# Autodesk Inventor assembly: x_motor
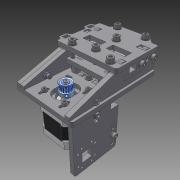
[picture p0: Inventor's stored thumbnail of the model, 180x180]
Saved by Autodesk Inventor 2014 (Build 180170000, 170)
## iProperties
Created: 2013-12-01
Part Number: x_motor
Document SubType Name: Assembly
Designer: buben
Author: buben
## Documents named in this file (23)
- C:\Users\buben\Documents\GitHub\bacon\inventor files\assemblies\x_motor.iam
- C:\Users\buben\Documents\GitHub\bacon\inventor files\printer parts\x_motor_back.ipt
- C:\Users\buben\Documents\GitHub\bacon\inventor files\printer parts\x_motor_wall_upper.ipt
- C:\Users\buben\Documents\GitHub\bacon\inventor files\printer parts\x_motor_middle.ipt
- C:\Users\buben\Documents\GitHub\bacon\inventor files\printer parts\x_motor_smooth_rod_spacer.ipt
- C:\Users\buben\Documents\GitHub\bacon\inventor files\3rd party components\linear_bearing_8\Imported Components\LU8MM\LU8MM.iam
- C:\Users\buben\Documents\GitHub\bacon\inventor files\printer parts\x_motor_top.ipt
- C:\Users\buben\Documents\GitHub\bacon\inventor files\utils\washer_m5.ipt
- C:\Users\buben\Documents\Inventor\Content Center Files\R2014\en-US\ISO 4762(2)\ISO 4762 - M5 x 45ISO.ipt
- C:\Users\buben\Documents\Inventor\Content Center Files\R2014\en-US\ISO 7040\ISO 7040 - M5.ipt
- C:\Users\buben\Documents\GitHub\bacon\inventor files\printer parts\x_motor_wall_lower.ipt
- C:\Users\buben\Documents\GitHub\bacon\inventor files\printer parts\x_motor_lower_nut_stop.ipt
- C:\Users\buben\Documents\GitHub\bacon\inventor files\utils\washer_m4.ipt
- C:\Users\buben\Documents\Inventor\Content Center Files\R2014\en-US\ISO 4762(2)\ISO 4762 - M4 x 20ISO.ipt
- C:\Users\buben\Documents\Inventor\Content Center Files\R2014\en-US\ISO 7040\ISO 7040 - M4.ipt
- C:\Users\buben\Documents\GitHub\bacon\inventor files\printer parts\x_motor_upper_nut_stop.ipt
- C:\Users\buben\Documents\Inventor\Content Center Files\R2014\en-US\ISO 4032(2)\ISO 4032 - M5ISO.ipt
- C:\Users\buben\Documents\GitHub\bacon\inventor files\printer parts\x_motor_cable_mount.ipt
- C:\Users\buben\Documents\GitHub\bacon\inventor files\printer parts\x_motor_cable_mount_brace.ipt
- C:\Users\buben\Documents\GitHub\bacon\inventor files\printer parts\motor_spacer.ipt
- C:\Users\buben\Documents\GitHub\bacon\inventor files\3rd party components\nema_17_stepper\Imported Components\NEMA 17 with T5 Pulley\NEMA 17 with T5 Pulley.iam
- C:\Users\buben\Documents\Inventor\Content Center Files\R2014\en-US\ISO 4762(2)\ISO 4762 - M3 x 20ISO.ipt
- C:\Users\buben\Documents\GitHub\bacon\inventor files\utils\washer_m3.ipt
## Components (73 placed, 22 different names)
1. x_motor_back:1 — Flush:1, Mate:1, Flush:2, Mate:2, Mate:3, Mate:4, Mate:8, Mate:9, Mate:10, Mate:11, Mate:12, Mate:13, Mate:35, Mate:36, Mate:37, Mate:38, Mate:39, Mate:40, Mate:59, Mate:60, Mate:61, Mate:77, Mate:103, Mate:104, Mate:105, Mate:109, Mate:110, Mate:113, Mate:114, Mate:130, Tangent:1, Tangent:2, Mate:131, Mate:132, Mate:133, Mate:134, Mate:139
2. x_motor_wall_upper:1 — Mate:2, Mate:3, Mate:4, Mate:5, Mate:6, Mate:7, Mate:20, Mate:21, Mate:78, Flush:3, Mate:85, Mate:100, Mate:101
3. x_motor_middle:1 — Mate:5, Mate:6, Mate:7, Mate:14, Mate:15, Mate:16, Mate:17, Mate:18, Mate:19, Mate:62, Mate:64
4. x_motor_smooth_rod_spacer:1 — Mate:8, Mate:9, Mate:10
5. x_motor_smooth_rod_spacer:2 — Mate:11, Mate:12, Mate:13
6. LU8MM:1 [sub-assembly] — Mate:14, Mate:15, Mate:18
7. LU8MM:2 [sub-assembly] — Mate:16, Mate:17, Mate:19, Mate:22
8. x_motor_top:1 — Mate:20, Mate:21, Mate:22, Mate:23, Mate:24, Mate:25, Mate:26, Mate:27, Mate:28, Mate:29, Mate:30, Mate:31, Mate:32, Mate:33, Mate:34
9. CSN 02 1702 B B 5,3:1 — Mate:26, Mate:31, Insert:1
10. CSN 02 1702 B B 5,3:2 — Mate:24, Mate:34, Insert:5
11. CSN 02 1702 B B 5,3:3 — Mate:23, Mate:32, Insert:6
12. CSN 02 1702 B B 5,3:4 — Mate:25, Mate:33, Insert:4
13. CSN 02 1702 B B 5,3:5 — Mate:27, Mate:29, Insert:3
14. CSN 02 1702 B B 5,3:6 — Mate:28, Mate:30, Insert:2
15. ISO 4762 M5 x 45:1 — Insert:5, Mate:45, Mate:48
16. ISO 4762 M5 x 45:2 — Insert:4, Mate:44, Mate:52
17. ISO 4762 M5 x 45:3 — Insert:3, Mate:41, Mate:56
18. ISO 4762 M5 x 45:4 — Insert:2, Mate:42, Mate:54
19. ISO 4762 M5 x 45:5 — Insert:1, Mate:43, Mate:58
20. ISO 4762 M5 x 45:6 — Insert:6, Mate:46, Mate:50
21. CSN 02 1702 B B 5,3:7 — Mate:40, Mate:41, Mate:55
22. CSN 02 1702 B B 5,3:8 — Mate:39, Mate:42, Mate:53
23. CSN 02 1702 B B 5,3:9 — Mate:38, Mate:43, Mate:57
24. CSN 02 1702 B B 5,3:10 — Mate:37, Mate:44, Mate:51
25. CSN 02 1702 B B 5,3:11 — Mate:36, Mate:46, Mate:49
26. CSN 02 1702 B B 5,3:12 — Mate:35, Mate:45, Mate:47
27. DIN EN ISO 7040 M5:1 — Mate:57, Mate:58
28. DIN EN ISO 7040 M5:2 — Mate:55, Mate:56
29. DIN EN ISO 7040 M5:3 — Mate:53, Mate:54
30. DIN EN ISO 7040 M5:4 — Mate:51, Mate:52
31. DIN EN ISO 7040 M5:5 — Mate:49, Mate:50
32. DIN EN ISO 7040 M5:6 — Mate:47, Mate:48
33. x_motor_wall_lower:1 — Mate:59, Mate:60, Mate:61, Mate:63, Mate:69, Mate:70, Mate:71, Mate:72, Mate:97, Mate:98
34. x_motor_lower_nut_stop:1 — Mate:62, Mate:63, Mate:64, Mate:65, Mate:66, Mate:67, Mate:68, Mate:99
35. CSN 02 1702 B B 4,3:1 — Mate:65, Mate:66, Mate:75
36. CSN 02 1702 B B 4,3:2 — Mate:67, Mate:68, Mate:73
37. CSN 02 1702 B B 4,3:3 — Mate:69, Mate:71, Insert:7
38. CSN 02 1702 B B 4,3:4 — Mate:70, Mate:72, Insert:8
39. ISO 4762 M4 x 20:1 — Insert:8, Mate:76
40. ISO 4762 M4 x 20:4 — Insert:9, Mate:86, Mate:88
41. ISO 4762 M4 x 20:5 — Insert:7, Mate:74
42. DIN EN ISO 7040 M4:1 — Mate:73, Mate:74
43. DIN EN ISO 7040 M4:3 — Mate:87, Mate:88
44. DIN EN ISO 7040 M4:4 — Mate:75, Mate:76
45. x_motor_upper_nut_stop:1 — Mate:77, Mate:78, Flush:3, Mate:81, Mate:82, Mate:102
46. CSN 02 1702 B B 4,3:7 — Mate:81, Mate:82, Insert:9
47. CSN 02 1702 B B 4,3:8 — Mate:85, Mate:86, Mate:87
48. ISO 4032 M5:1 — Mate:97, Mate:98, Mate:99
49. ISO 4032 M5:2 — Mate:100, Mate:101, Mate:102
50. x_motor_cable_mount:1 — Mate:103, Mate:104, Mate:105, Mate:111, Mate:112, Mate:115, Mate:140, Mate:141
51. CSN 02 1702 B B 4,3:11 — Mate:109, Mate:110, Insert:12
52. CSN 02 1702 B B 4,3:12 — Mate:113, Mate:114, Insert:14
53. CSN 02 1702 B B 4,3:13 — Mate:111, Mate:112, Insert:13
54. CSN 02 1702 B B 4,3:14 — Mate:120, Mate:123, Mate:142
55. CSN 02 1702 B B 4,3:15 — Mate:118, Mate:121, Mate:143
56. CSN 02 1702 B B 4,3:16 — Mate:115, Mate:116, Mate:125
57. ISO 4762 M4 x 20:6 — Insert:12, Mate:116, Mate:126
58. ISO 4762 M4 x 20:7 — Insert:13, Mate:120, Mate:124
59. ISO 4762 M4 x 20:8 — Insert:14, Mate:118, Mate:122
60. DIN EN ISO 7040 M4:6 — Mate:121, Mate:122
61. DIN EN ISO 7040 M4:7 — Mate:123, Mate:124
62. DIN EN ISO 7040 M4:8 — Mate:125, Mate:126
63. motor_spacer:1 — Mate:127, Mate:128, Mate:129, Mate:130, Tangent:1, Tangent:2, Mate:135, Mate:136, Mate:137, Mate:138
64. NEMA 17 with T5 Pulley:1 [sub-assembly] — Mate:127, Mate:128, Mate:129
65. ISO 4762 M3 x 20:1 — Insert:16, Mate:137
66. ISO 4762 M3 x 20:2 — Insert:18, Mate:138
67. ISO 4762 M3 x 20:3 — Insert:17, Mate:135
68. ISO 4762 M3 x 20:4 — Insert:15, Mate:136
69. CSN 02 1702 B B 3,2:1 — Mate:134, Insert:17
70. CSN 02 1702 B B 3,2:2 — Mate:133, Insert:18
71. CSN 02 1702 B B 3,2:3 — Mate:132, Insert:15
72. CSN 02 1702 B B 3,2:4 — Mate:131, Insert:16
73. x_motor_cable_mount_brace:1 — Mate:139, Mate:140, Mate:141, Mate:142, Mate:143
## Relationships (147: Mate 126, Insert 16, Flush 3, Tangent 2)
- Flush:1: x_motor_back:1
- Mate:1: x_motor_back:1
- Flush:2: x_motor_back:1
- Mate:2: x_motor_back:1 ↔ x_motor_wall_upper:1
- Mate:3: x_motor_back:1 ↔ x_motor_wall_upper:1
- Mate:4: x_motor_back:1 ↔ x_motor_wall_upper:1
- Mate:5: x_motor_wall_upper:1 ↔ x_motor_middle:1
- Mate:6: x_motor_wall_upper:1 ↔ x_motor_middle:1
- Mate:7: x_motor_wall_upper:1 ↔ x_motor_middle:1
- Mate:8: x_motor_back:1 ↔ x_motor_smooth_rod_spacer:1
- Mate:9: x_motor_back:1 ↔ x_motor_smooth_rod_spacer:1
- Mate:10: x_motor_back:1 ↔ x_motor_smooth_rod_spacer:1
- Mate:11: x_motor_back:1 ↔ x_motor_smooth_rod_spacer:2
- Mate:12: x_motor_back:1 ↔ x_motor_smooth_rod_spacer:2
- Mate:13: x_motor_back:1 ↔ x_motor_smooth_rod_spacer:2
- Mate:14 (7.5 mm): x_motor_middle:1 ↔ LU8MM:1
- Mate:15 (7.5 mm): x_motor_middle:1 ↔ LU8MM:1
- Mate:16 (7.5 mm): x_motor_middle:1 ↔ LU8MM:2
- Mate:17 (7.5 mm): x_motor_middle:1 ↔ LU8MM:2
- Mate:18 (0.5 mm): x_motor_middle:1 ↔ LU8MM:1
- Mate:19 (0.5 mm): x_motor_middle:1 ↔ LU8MM:2
- Mate:20: x_motor_wall_upper:1 ↔ x_motor_top:1
- Mate:21: x_motor_wall_upper:1 ↔ x_motor_top:1
- Mate:22 (7.5 mm): LU8MM:2 ↔ x_motor_top:1
- Mate:23: x_motor_top:1 ↔ CSN 02 1702 B B 5,3:3
- Mate:24: x_motor_top:1 ↔ CSN 02 1702 B B 5,3:2
- Mate:25: x_motor_top:1 ↔ CSN 02 1702 B B 5,3:4
- Mate:26: x_motor_top:1 ↔ CSN 02 1702 B B 5,3:1
- Mate:27: x_motor_top:1 ↔ CSN 02 1702 B B 5,3:5
- Mate:28: x_motor_top:1 ↔ CSN 02 1702 B B 5,3:6
- Mate:29: x_motor_top:1 ↔ CSN 02 1702 B B 5,3:5
- Mate:30: x_motor_top:1 ↔ CSN 02 1702 B B 5,3:6
- Mate:31: x_motor_top:1 ↔ CSN 02 1702 B B 5,3:1
- Mate:32: x_motor_top:1 ↔ CSN 02 1702 B B 5,3:3
- Mate:33: x_motor_top:1 ↔ CSN 02 1702 B B 5,3:4
- Mate:34: x_motor_top:1 ↔ CSN 02 1702 B B 5,3:2
- Insert:1: CSN 02 1702 B B 5,3:1 ↔ ISO 4762 M5 x 45:5
- Insert:2: CSN 02 1702 B B 5,3:6 ↔ ISO 4762 M5 x 45:4
- Insert:3: CSN 02 1702 B B 5,3:5 ↔ ISO 4762 M5 x 45:3
- Insert:4: CSN 02 1702 B B 5,3:4 ↔ ISO 4762 M5 x 45:2
- Insert:5: CSN 02 1702 B B 5,3:2 ↔ ISO 4762 M5 x 45:1
- Insert:6: CSN 02 1702 B B 5,3:3 ↔ ISO 4762 M5 x 45:6
- Mate:35: x_motor_back:1 ↔ CSN 02 1702 B B 5,3:12
- Mate:36: x_motor_back:1 ↔ CSN 02 1702 B B 5,3:11
- Mate:37: x_motor_back:1 ↔ CSN 02 1702 B B 5,3:10
- Mate:38: x_motor_back:1 ↔ CSN 02 1702 B B 5,3:9
- Mate:39: x_motor_back:1 ↔ CSN 02 1702 B B 5,3:8
- Mate:40: x_motor_back:1 ↔ CSN 02 1702 B B 5,3:7
- Mate:41: ISO 4762 M5 x 45:3 ↔ CSN 02 1702 B B 5,3:7
- Mate:42: ISO 4762 M5 x 45:4 ↔ CSN 02 1702 B B 5,3:8
- Mate:43: ISO 4762 M5 x 45:5 ↔ CSN 02 1702 B B 5,3:9
- Mate:44: ISO 4762 M5 x 45:2 ↔ CSN 02 1702 B B 5,3:10
- Mate:45: ISO 4762 M5 x 45:1 ↔ CSN 02 1702 B B 5,3:12
- Mate:46: ISO 4762 M5 x 45:6 ↔ CSN 02 1702 B B 5,3:11
- Mate:47: CSN 02 1702 B B 5,3:12 ↔ DIN EN ISO 7040 M5:6
- Mate:48: ISO 4762 M5 x 45:1 ↔ DIN EN ISO 7040 M5:6
- Mate:49: CSN 02 1702 B B 5,3:11 ↔ DIN EN ISO 7040 M5:5
- Mate:50: ISO 4762 M5 x 45:6 ↔ DIN EN ISO 7040 M5:5
- Mate:51: CSN 02 1702 B B 5,3:10 ↔ DIN EN ISO 7040 M5:4
- Mate:52: ISO 4762 M5 x 45:2 ↔ DIN EN ISO 7040 M5:4
- Mate:53: CSN 02 1702 B B 5,3:8 ↔ DIN EN ISO 7040 M5:3
- Mate:54: ISO 4762 M5 x 45:4 ↔ DIN EN ISO 7040 M5:3
- Mate:55: CSN 02 1702 B B 5,3:7 ↔ DIN EN ISO 7040 M5:2
- Mate:56: ISO 4762 M5 x 45:3 ↔ DIN EN ISO 7040 M5:2
- Mate:57: CSN 02 1702 B B 5,3:9 ↔ DIN EN ISO 7040 M5:1
- Mate:58: ISO 4762 M5 x 45:5 ↔ DIN EN ISO 7040 M5:1
- Mate:59: x_motor_back:1 ↔ x_motor_wall_lower:1
- Mate:60: x_motor_back:1 ↔ x_motor_wall_lower:1
- Mate:61: x_motor_back:1 ↔ x_motor_wall_lower:1
- Mate:62: x_motor_middle:1 ↔ x_motor_lower_nut_stop:1
- Mate:63: x_motor_wall_lower:1 ↔ x_motor_lower_nut_stop:1
- Mate:64: x_motor_middle:1 ↔ x_motor_lower_nut_stop:1
- Mate:65: x_motor_lower_nut_stop:1 ↔ CSN 02 1702 B B 4,3:1
- Mate:66: x_motor_lower_nut_stop:1 ↔ CSN 02 1702 B B 4,3:1
- Mate:67: x_motor_lower_nut_stop:1 ↔ CSN 02 1702 B B 4,3:2
- Mate:68: x_motor_lower_nut_stop:1 ↔ CSN 02 1702 B B 4,3:2
- Mate:69: x_motor_wall_lower:1 ↔ CSN 02 1702 B B 4,3:3
- Mate:70: x_motor_wall_lower:1 ↔ CSN 02 1702 B B 4,3:4
- Mate:71: x_motor_wall_lower:1 ↔ CSN 02 1702 B B 4,3:3
- Mate:72: x_motor_wall_lower:1 ↔ CSN 02 1702 B B 4,3:4
- Insert:7: CSN 02 1702 B B 4,3:3 ↔ ISO 4762 M4 x 20:5
- Insert:8: CSN 02 1702 B B 4,3:4 ↔ ISO 4762 M4 x 20:1
- Mate:73: CSN 02 1702 B B 4,3:2 ↔ DIN EN ISO 7040 M4:1
- Mate:74: ISO 4762 M4 x 20:5 ↔ DIN EN ISO 7040 M4:1
- Mate:75: CSN 02 1702 B B 4,3:1 ↔ DIN EN ISO 7040 M4:4
- Mate:76: ISO 4762 M4 x 20:1 ↔ DIN EN ISO 7040 M4:4
- Mate:77: x_motor_back:1 ↔ x_motor_upper_nut_stop:1
- Mate:78: x_motor_wall_upper:1 ↔ x_motor_upper_nut_stop:1
- Flush:3: x_motor_wall_upper:1 ↔ x_motor_upper_nut_stop:1
- Mate:81: x_motor_upper_nut_stop:1 ↔ CSN 02 1702 B B 4,3:7
- Mate:82: x_motor_upper_nut_stop:1 ↔ CSN 02 1702 B B 4,3:7
- Insert:9: ISO 4762 M4 x 20:4 ↔ CSN 02 1702 B B 4,3:7
- Mate:85: x_motor_wall_upper:1 ↔ CSN 02 1702 B B 4,3:8
- Mate:86: ISO 4762 M4 x 20:4 ↔ CSN 02 1702 B B 4,3:8
- Mate:87: DIN EN ISO 7040 M4:3 ↔ CSN 02 1702 B B 4,3:8
- Mate:88: ISO 4762 M4 x 20:4 ↔ DIN EN ISO 7040 M4:3
- Mate:97: x_motor_wall_lower:1 ↔ ISO 4032 M5:1
- Mate:98: x_motor_wall_lower:1 ↔ ISO 4032 M5:1
- Mate:99: x_motor_lower_nut_stop:1 ↔ ISO 4032 M5:1
- Mate:100: x_motor_wall_upper:1 ↔ ISO 4032 M5:2
- Mate:101: x_motor_wall_upper:1 ↔ ISO 4032 M5:2
- Mate:102: x_motor_upper_nut_stop:1 ↔ ISO 4032 M5:2
- Mate:103: x_motor_back:1 ↔ x_motor_cable_mount:1
- Mate:104: x_motor_back:1 ↔ x_motor_cable_mount:1
- Mate:105: x_motor_back:1 ↔ x_motor_cable_mount:1
- Mate:109: x_motor_back:1 ↔ CSN 02 1702 B B 4,3:11
- Mate:110: x_motor_back:1 ↔ CSN 02 1702 B B 4,3:11
- Insert:12: CSN 02 1702 B B 4,3:11 ↔ ISO 4762 M4 x 20:6
- Mate:111: x_motor_cable_mount:1 ↔ CSN 02 1702 B B 4,3:13
- Mate:112: x_motor_cable_mount:1 ↔ CSN 02 1702 B B 4,3:13
- Mate:113: x_motor_back:1 ↔ CSN 02 1702 B B 4,3:12
- Mate:114: x_motor_back:1 ↔ CSN 02 1702 B B 4,3:12
- Insert:13: CSN 02 1702 B B 4,3:13 ↔ ISO 4762 M4 x 20:7
- Insert:14: CSN 02 1702 B B 4,3:12 ↔ ISO 4762 M4 x 20:8
- Mate:115: x_motor_cable_mount:1 ↔ CSN 02 1702 B B 4,3:16
- Mate:116: CSN 02 1702 B B 4,3:16 ↔ ISO 4762 M4 x 20:6
- Mate:118: CSN 02 1702 B B 4,3:15 ↔ ISO 4762 M4 x 20:8
- Mate:120: CSN 02 1702 B B 4,3:14 ↔ ISO 4762 M4 x 20:7
- Mate:121: CSN 02 1702 B B 4,3:15 ↔ DIN EN ISO 7040 M4:6
- Mate:122: ISO 4762 M4 x 20:8 ↔ DIN EN ISO 7040 M4:6
- Mate:123: CSN 02 1702 B B 4,3:14 ↔ DIN EN ISO 7040 M4:7
- Mate:124: ISO 4762 M4 x 20:7 ↔ DIN EN ISO 7040 M4:7
- Mate:125: CSN 02 1702 B B 4,3:16 ↔ DIN EN ISO 7040 M4:8
- Mate:126: ISO 4762 M4 x 20:6 ↔ DIN EN ISO 7040 M4:8
- Mate:127: motor_spacer:1 ↔ NEMA 17 with T5 Pulley:1
- Mate:128: motor_spacer:1 ↔ NEMA 17 with T5 Pulley:1
- Mate:129: motor_spacer:1 ↔ NEMA 17 with T5 Pulley:1
- Mate:130: x_motor_back:1 ↔ motor_spacer:1
- Tangent:1: x_motor_back:1 ↔ motor_spacer:1
- Tangent:2: x_motor_back:1 ↔ motor_spacer:1
- Mate:131: x_motor_back:1 ↔ CSN 02 1702 B B 3,2:4
- Mate:132: x_motor_back:1 ↔ CSN 02 1702 B B 3,2:3
- Mate:133: x_motor_back:1 ↔ CSN 02 1702 B B 3,2:2
- Mate:134: x_motor_back:1 ↔ CSN 02 1702 B B 3,2:1
- Insert:15: ISO 4762 M3 x 20:4 ↔ CSN 02 1702 B B 3,2:3
- Insert:16: ISO 4762 M3 x 20:1 ↔ CSN 02 1702 B B 3,2:4
- Insert:17: ISO 4762 M3 x 20:3 ↔ CSN 02 1702 B B 3,2:1
- Insert:18: ISO 4762 M3 x 20:2 ↔ CSN 02 1702 B B 3,2:2
- Mate:135: motor_spacer:1 ↔ ISO 4762 M3 x 20:3
- Mate:136: motor_spacer:1 ↔ ISO 4762 M3 x 20:4
- Mate:137: motor_spacer:1 ↔ ISO 4762 M3 x 20:1
- Mate:138: motor_spacer:1 ↔ ISO 4762 M3 x 20:2
- Mate:139: x_motor_back:1 ↔ x_motor_cable_mount_brace:1
- Mate:140: x_motor_cable_mount:1 ↔ x_motor_cable_mount_brace:1
- Mate:141: x_motor_cable_mount:1 ↔ x_motor_cable_mount_brace:1
- Mate:142: CSN 02 1702 B B 4,3:14 ↔ x_motor_cable_mount_brace:1
- Mate:143: CSN 02 1702 B B 4,3:15 ↔ x_motor_cable_mount_brace:1
